# Autodesk Inventor assembly: 組合1
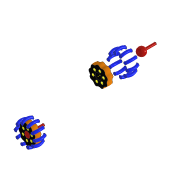
[picture p0: Inventor's stored thumbnail of the model, 180x180]
Saved by Autodesk Inventor 2022 (Build 260153000, 153)
## iProperties
Created: 2023-10-11
Part Number: 組合1
Document SubType Name: Assembly
Designer: JOU
Author: JOU
## Documents named in this file (4)
- C:\Users\JOU\Desktop\git\Special-project\接觸解析器練習資料夾\接觸解析器練習資料夾\Cycloidal Gear\ball\組合1.iam
- C:\Users\JOU\Desktop\git\Special-project\接觸解析器練習資料夾\接觸解析器練習資料夾\Cycloidal Gear\ball\Roller_Gear.ipt
- C:\Users\JOU\Desktop\git\Special-project\接觸解析器練習資料夾\接觸解析器練習資料夾\Cycloidal Gear\ball\Input_Shaft.ipt
- C:\Users\JOU\Desktop\git\Special-project\接觸解析器練習資料夾\接觸解析器練習資料夾\Cycloidal Gear\ball\Cycloid_Gear.ipt
## Components (6 placed, 3 different names)
1. Roller_Gear:1 — 貼合:1
2. Input_Shaft:1 — 貼合:1, 相切:1
3. Cycloid_Gear:1 — 相切:1
4. Cycloid_Gear:2 — 貼合:2
5. Roller_Gear:2 — 貼合:3
6. Input_Shaft:2 — 貼合:2, 貼合:3
## Relationships (4: Mate 3, Tangent 1)
- 貼合:1 [Mate]: Roller_Gear:1 ↔ Input_Shaft:1
- 相切:1 [Tangent]: Input_Shaft:1 ↔ Cycloid_Gear:1
- 貼合:2 [Mate]: Cycloid_Gear:2 ↔ Input_Shaft:2
- 貼合:3 [Mate]: Roller_Gear:2 ↔ Input_Shaft:2
